# Autodesk Inventor assembly: Draft_01_1
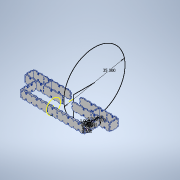
[picture p0: Inventor's stored thumbnail of the model, 180x180]
Saved by Autodesk Inventor 2021 (Build 250183000, 183)
## iProperties
Created: 2021-03-05
Part Number: Draft_01_1
Document SubType Name: Assembly
Designer: M3rob
Mass: 56682.1 g
Surface Area: 31959.2 cm^2
Volume: 19618.1 cm^3
Density: 2.88927 g/cm^3
Author: M3rob
## Documents named in this file (9)
- C:\Users\M3rob\Documents\GrabCAD\FireBird 250 Pound Gaming Machine\Drafts\FrameDrafts\Draft_01_1\Draft_01_1.iam
- C:\Users\M3rob\Documents\GrabCAD\FireBird 250 Pound Gaming Machine\Drafts\FrameDrafts\Draft_01_1\BackWallFrame.ipt
- C:\Users\M3rob\Documents\GrabCAD\FireBird 250 Pound Gaming Machine\Drafts\FrameDrafts\Draft_01_1\DriveFrame.ipt
- C:\Users\M3rob\Documents\GrabCAD\FireBird 250 Pound Gaming Machine\Drafts\FrameDrafts\Draft_01_1\NeckFrame.ipt
- C:\Users\M3rob\Documents\GrabCAD\FireBird 250 Pound Gaming Machine\Drafts\FrameDrafts\Draft_01_1\FrontFrame.ipt
- C:\Users\M3rob\Documents\GrabCAD\FireBird 250 Pound Gaming Machine\Drafts\FrameDrafts\Draft_01_1\SmallSideFrame.ipt
- C:\Users\M3rob\Documents\GrabCAD\FireBird 250 Pound Gaming Machine\Drafts\FrameDrafts\Draft_01_1\AluminumTopPlate.ipt
- C:\Users\M3rob\Documents\GrabCAD\FireBird 250 Pound Gaming Machine\Drafts\FrameDrafts\Draft_01_1\ThiccUpright.ipt
- C:\Users\M3rob\Documents\GrabCAD\FireBird 250 Pound Gaming Machine\Drafts\FrameDrafts\Draft_01_1\MockupWheel.ipt
## Components (19 placed, 8 different names)
1. BackWallFrame:1 — Flush:1, Mate:1, Mate:2, Mate:3, Mate:4, Flush:2, Mate:5, Mate:6, Mate:7, Mate:8, Mate:9, Mate:10
2. DriveFrame:1 — Mate:3, Mate:4, Flush:2, Insert:1
3. DriveFrame:2 — Flush:1, Mate:1, Mate:2, Mate:13, Insert:2
4. NeckFrame:1 — Mate:5, Mate:6, Mate:7, Mate:11, Mate:12, Mate:14, Mate:15, Mate:16, Mate:40, Mate:41, Mate:42
5. NeckFrame:2 — Mate:8, Mate:9, Mate:10, Mate:17, Mate:18, Mate:19, Mate:20, Mate:21, Mate:22, Mate:36, Mate:37, Mate:38, Mate:43
6. FrontFrame:1 — Mate:11, Mate:12, Mate:16, Mate:24, Mate:25, Mate:26, Mate:27, Mate:28, Flush:3
7. FrontFrame:2 — Mate:20, Mate:21, Mate:22, Mate:29, Mate:32, Mate:34, Mate:35
8. FrontFrame:3 — Mate:13, Mate:14, Mate:15, Mate:23
9. FrontFrame:4 — Mate:17, Mate:18, Mate:19, Mate:30, Mate:31, Mate:33, Flush:4
10. SmallSideFrame:1 — Mate:23, Mate:24, Mate:25
11. SmallSideFrame:2 — Mate:26, Mate:27, Mate:28
12. SmallSideFrame:3 — Mate:32, Mate:33, Mate:34, Mate:35
13. SmallSideFrame:4 — Mate:29, Mate:30, Mate:31, Flush:5
14. AluminumTopPlate:1 — Flush:3
15. AluminumTopPlate:2 — Flush:4, Flush:5, Mate:36
16. ThiccUpright:1 — Mate:40, Mate:41, Mate:42
17. ThiccUpright:2 — Mate:37, Mate:38, Mate:43
18. MockupWheel:1 — Insert:1
19. MockupWheel:2 — Insert:2
## Relationships (49: Mate 42, Flush 5, Insert 2)
- Flush:1: BackWallFrame:1 ↔ DriveFrame:2
- Mate:1: BackWallFrame:1 ↔ DriveFrame:2
- Mate:2: BackWallFrame:1 ↔ DriveFrame:2
- Mate:3: BackWallFrame:1 ↔ DriveFrame:1
- Mate:4: BackWallFrame:1 ↔ DriveFrame:1
- Flush:2: BackWallFrame:1 ↔ DriveFrame:1
- Mate:5: BackWallFrame:1 ↔ NeckFrame:1
- Mate:6: BackWallFrame:1 ↔ NeckFrame:1
- Mate:7: BackWallFrame:1 ↔ NeckFrame:1
- Mate:8: BackWallFrame:1 ↔ NeckFrame:2
- Mate:9: BackWallFrame:1 ↔ NeckFrame:2
- Mate:10: BackWallFrame:1 ↔ NeckFrame:2
- Mate:11: NeckFrame:1 ↔ FrontFrame:1
- Mate:12: NeckFrame:1 ↔ FrontFrame:1
- Mate:13: DriveFrame:2 ↔ FrontFrame:3
- Mate:14: NeckFrame:1 ↔ FrontFrame:3
- Mate:15: NeckFrame:1 ↔ FrontFrame:3
- Mate:16: NeckFrame:1 ↔ FrontFrame:1
- Mate:17: NeckFrame:2 ↔ FrontFrame:4
- Mate:18: NeckFrame:2 ↔ FrontFrame:4
- Mate:19: NeckFrame:2 ↔ FrontFrame:4
- Mate:20: NeckFrame:2 ↔ FrontFrame:2
- Mate:21: NeckFrame:2 ↔ FrontFrame:2
- Mate:22: NeckFrame:2 ↔ FrontFrame:2
- Mate:23: FrontFrame:3 ↔ SmallSideFrame:1
- Mate:24: FrontFrame:1 ↔ SmallSideFrame:1
- Mate:25: FrontFrame:1 ↔ SmallSideFrame:1
- Mate:26: FrontFrame:1 ↔ SmallSideFrame:2
- Mate:27: FrontFrame:1 ↔ SmallSideFrame:2
- Mate:28: FrontFrame:1 ↔ SmallSideFrame:2
- Mate:29: FrontFrame:2 ↔ SmallSideFrame:4
- Mate:30: FrontFrame:4 ↔ SmallSideFrame:4
- Mate:31: FrontFrame:4 ↔ SmallSideFrame:4
- Mate:32: FrontFrame:2 ↔ SmallSideFrame:3
- Mate:33: FrontFrame:4 ↔ SmallSideFrame:3
- Mate:34: FrontFrame:2 ↔ SmallSideFrame:3
- Mate:35: FrontFrame:2 ↔ SmallSideFrame:3
- Flush:3: FrontFrame:1 ↔ AluminumTopPlate:1
- Flush:4: FrontFrame:4 ↔ AluminumTopPlate:2
- Flush:5: SmallSideFrame:4 ↔ AluminumTopPlate:2
- Mate:36: NeckFrame:2 ↔ AluminumTopPlate:2
- Mate:37: NeckFrame:2 ↔ ThiccUpright:2
- Mate:38: NeckFrame:2 ↔ ThiccUpright:2
- Mate:40: NeckFrame:1 ↔ ThiccUpright:1
- Mate:41: NeckFrame:1 ↔ ThiccUpright:1
- Mate:42: NeckFrame:1 ↔ ThiccUpright:1
- Insert:1: DriveFrame:1 ↔ MockupWheel:1
- Insert:2: DriveFrame:2 ↔ MockupWheel:2
- Mate:43: NeckFrame:2 ↔ ThiccUpright:2
